# Autodesk Inventor assembly: Jack Assembly
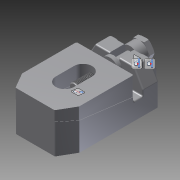
[picture p0: Inventor's stored thumbnail of the model, 180x180]
Saved by Autodesk Inventor 2015 (Build 190159000, 159)
## iProperties
Created: 2018-02-22
Part Number: Jack Assembly
Document SubType Name: Assembly
Designer: Administrator
Author: Administrator
## Documents named in this file (4)
- L:\IED 9th\7.4 Jack\Jack Assembly.iam
- L:\IED 9th\7.4 Jack\Base.ipt
- L:\IED 9th\7.4 Jack\Wedge.ipt
- L:\IED 9th\7.4 Jack\Wedge_Screw.ipt
## Components (3 placed, 3 different names)
1. Base:1 — Tangent:1, Tangent:2, Mate:1, Mate:2, Flush:1
2. Wedge:1 — Mate:2, Mate:3, Flush:1
3. Wedge_Screw:1 — Tangent:1, Tangent:2, Mate:1, Mate:3
## Relationships (6: Mate 3, Tangent 2, Flush 1)
- Tangent:1: Base:1 ↔ Wedge_Screw:1
- Tangent:2: Base:1 ↔ Wedge_Screw:1
- Mate:1: Base:1 ↔ Wedge_Screw:1
- Mate:2: Base:1 ↔ Wedge:1
- Mate:3: Wedge:1 ↔ Wedge_Screw:1
- Flush:1: Base:1 ↔ Wedge:1
